# Autodesk Inventor assembly: Hand
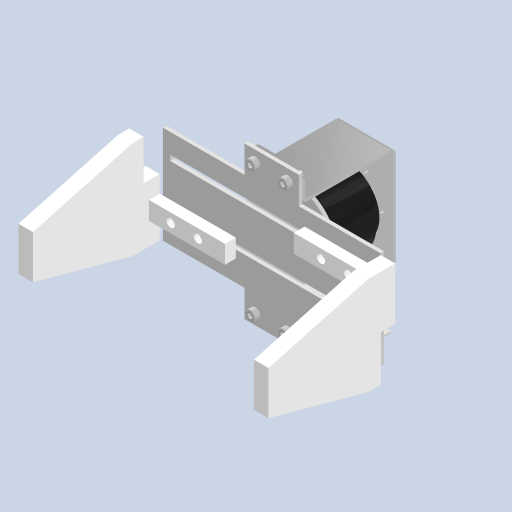
[picture p0: Inventor's stored thumbnail of the model, 512x512]
Saved by Autodesk Inventor 2023 (Build 270158000, 158)
## iProperties
Created: 2024-11-27
Part Number: Hand
Document SubType Name: Assembly
Designer: kiyo
Mass: 142.009 g
Surface Area: 718.919 cm^2
Volume: 132.865 cm^3
Density: 1.06882 g/cm^3
Author: kiyo
## Documents named in this file (14)
- D:\GitHub\inventor\syu-si\OfficeRobot\Hand\Hand.iam
- D:\GitHub\inventor\syu-si\OfficeRobot\ReadyMade\Steadywin\GIM3505-8_with-driver.ipt
- D:\GitHub\inventor\syu-si\OfficeRobot\ReadyMade\Screw\GFM-0304-03.ipt
- D:\GitHub\inventor\syu-si\OfficeRobot\ReadyMade\Screw\FB-305530.ipt
- D:\GitHub\inventor\syu-si\OfficeRobot\Hand\motor-fixing.ipt
- D:\GitHub\inventor\syu-si\OfficeRobot\Hand\hand_box1.ipt
- D:\GitHub\inventor\syu-si\OfficeRobot\Hand\right-nail.ipt
- D:\GitHub\inventor\syu-si\OfficeRobot\Hand\left-nail.ipt
- D:\GitHub\inventor\syu-si\OfficeRobot\Hand\rackgear.ipt
- D:\GitHub\inventor\syu-si\OfficeRobot\Hand\hand-gear.ipt
- D:\GitHub\inventor\syu-si\OfficeRobot\ReadyMade\Screw\CBE3-8.ipt
- D:\GitHub\inventor\syu-si\OfficeRobot\ReadyMade\Screw\CSH-316L-M2_5-6.ipt
- D:\GitHub\inventor\syu-si\OfficeRobot\ReadyMade\Screw\CBE3-5.ipt
- D:\GitHub\inventor\syu-si\OfficeRobot\Hand\Old_hand_box2.ipt
## Components (35 placed, 13 different names)
1. GIM3505-8_with-driver:1 — 挿入:45, 挿入:46, 角度:1
2. left-nail:2
3. right-nail:2
4. hand_box1:1 — 挿入:65, 挿入:66, 挿入:67, 挿入:68, メイト:10, メイト:11
5. rackgear:4 — 挿入:59, 挿入:60, メイト:11
6. rackgear:3 — 挿入:57, 挿入:58, メイト:10
7. hand-gear
8. motor-fixing:1 — 挿入:45, 挿入:46, 挿入:69, 挿入:70, 挿入:71, 挿入:74, 挿入:75
9. Old_hand_box2:1 — 挿入:72, 挿入:73, 挿入:76, 角度:1
10. CSH-316L-M2_5-6:1
11. CSH-316L-M2_5-6:2
12. CSH-316L-M2_5-6:3
13. CSH-316L-M2_5-6:4 — 挿入:71
14. CSH-316L-M2_5-6:5 — 挿入:70
15. CSH-316L-M2_5-6:6 — 挿入:69
16. CBE3-5:1 — 挿入:66
17. CBE3-5:2 — 挿入:65
18. CBE3-5:3 — 挿入:68
19. CBE3-5:4 — 挿入:67
20. CBE3-5:5 — 挿入:72
21. CBE3-5:6 — 挿入:73
22. CBE3-8:1 — 挿入:59
23. CBE3-8:2 — 挿入:60
24. CBE3-8:3 — 挿入:58
25. CBE3-8:4 — 挿入:57
26. FB-305530:1
27. FB-305530:2
28. FB-305530:3
29. FB-305530:4
30. FB-305530:5 — 挿入:75
31. FB-305530:6 — 挿入:74, 挿入:76
32. GFM-0304-03:1
33. GFM-0304-03:2
34. GFM-0304-03:3
35. GFM-0304-03:4
## Relationships (45: Insert 36, Mate 6, Flush 2, Angle 1)
- [Insert]: GIM3505-8_with-driver:1 ↔ hand-gear
- [Mate] (0.05 mm): hand_box1:1 ↔ rackgear:3
- [Mate] (0.05 mm): hand_box1:1 ↔ rackgear:4
- [Insert]: left-nail:2 ↔ GFM-0304-03:1
- [Insert]: left-nail:2 ↔ GFM-0304-03:2
- [Insert]: rackgear:3 ↔ GFM-0304-03:2
- [Insert]: rackgear:3 ↔ GFM-0304-03:1
- [Mate]: hand_box1:1 ↔ GFM-0304-03:1
- [Insert]: right-nail:2 ↔ GFM-0304-03:3
- [Insert]: right-nail:2 ↔ GFM-0304-03:4
- [Mate]: hand_box1:1 ↔ GFM-0304-03:3
- [Insert]: rackgear:4 ↔ GFM-0304-03:3
- [Insert]: rackgear:4 ↔ GFM-0304-03:4
- [Insert]: right-nail:2 ↔ FB-305530:1
- [Insert]: right-nail:2 ↔ FB-305530:2
- [Insert]: left-nail:2 ↔ FB-305530:4
- [Insert]: left-nail:2 ↔ FB-305530:3
- [Flush] (60 mm): right-nail:2 ↔ hand_box1:1
- [Flush] (60 mm): left-nail:2 ↔ hand_box1:1
- [Insert]: hand-gear ↔ CSH-316L-M2_5-6:3
- [Insert]: hand-gear ↔ CSH-316L-M2_5-6:2
- [Insert]: hand-gear ↔ CSH-316L-M2_5-6:1
- 挿入:45 [Insert]: GIM3505-8_with-driver:1 ↔ motor-fixing:1
- 挿入:46 [Insert]: GIM3505-8_with-driver:1 ↔ motor-fixing:1
- [Insert]: hand_box1:1 ↔ Old_hand_box2:1
- [Insert]: hand_box1:1 ↔ Old_hand_box2:1
- 挿入:57 [Insert]: rackgear:3 ↔ CBE3-8:4
- 挿入:58 [Insert]: rackgear:3 ↔ CBE3-8:3
- 挿入:59 [Insert]: rackgear:4 ↔ CBE3-8:1
- 挿入:60 [Insert]: rackgear:4 ↔ CBE3-8:2
- 挿入:65 [Insert]: hand_box1:1 ↔ CBE3-5:2
- 挿入:66 [Insert]: hand_box1:1 ↔ CBE3-5:1
- 挿入:67 [Insert]: hand_box1:1 ↔ CBE3-5:4
- 挿入:68 [Insert]: hand_box1:1 ↔ CBE3-5:3
- 挿入:69 [Insert]: motor-fixing:1 ↔ CSH-316L-M2_5-6:6
- 挿入:70 [Insert]: motor-fixing:1 ↔ CSH-316L-M2_5-6:5
- 挿入:71 [Insert]: motor-fixing:1 ↔ CSH-316L-M2_5-6:4
- メイト:10 [Mate]: hand_box1:1 ↔ rackgear:3
- メイト:11 [Mate]: hand_box1:1 ↔ rackgear:4
- 挿入:72 [Insert]: Old_hand_box2:1 ↔ CBE3-5:5
- 挿入:73 [Insert]: Old_hand_box2:1 ↔ CBE3-5:6
- 挿入:74 [Insert]: motor-fixing:1 ↔ FB-305530:6
- 挿入:75 [Insert]: motor-fixing:1 ↔ FB-305530:5
- 挿入:76 [Insert]: Old_hand_box2:1 ↔ FB-305530:6
- 角度:1 [Angle] (0 deg): GIM3505-8_with-driver:1 ↔ Old_hand_box2:1
